# Autodesk Inventor assembly: Pogo_Set2
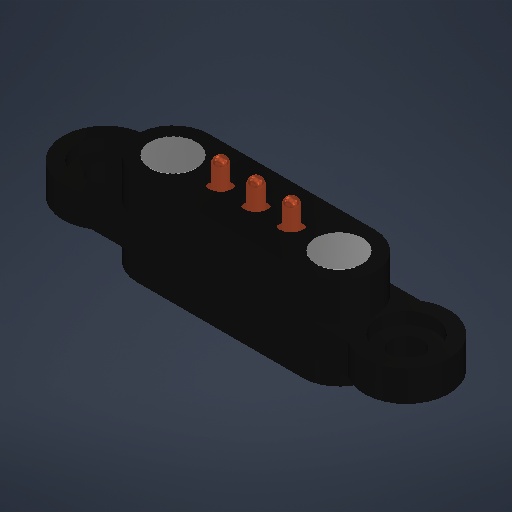
[picture p0: Inventor's stored thumbnail of the model, 512x512]
Saved by Autodesk Inventor 2026 (Build 300175000, 175)
## iProperties
Created: 2025-04-18
Part Number: Pogo_Set2
Document SubType Name: Assembly
Designer: ct_vi
Author: ct_vi
## Documents named in this file (5)
- C:\Users\ct_vi\Documents\Capstone_Research_3D_Files\Pogo_Set2.iam
- C:\Users\ct_vi\Documents\Capstone_Research_3D_Files\Pogo2.ipt
- C:\Users\ct_vi\Documents\Capstone_Research_3D_Files\Pogo_Pin2.ipt
- Pogo_Pin2.ipt
- C:\Users\ct_vi\Documents\Capstone_Research_3D_Files\Magnet_Pogo2.ipt
## Components (4 placed, 3 different names)
1. Pogo_Pin2:1 — Mate:1, Mate:2, Mate:3
2. Pogo2:2 — Mate:1, Mate:2, Mate:3, Mate:4, Mate:5, Flush:1, Flush:2
3. Magnet_Pogo2:1 — Mate:5, Flush:1
4. Magnet_Pogo2:2 — Mate:4, Flush:2
## Relationships (7: Mate 5, Flush 2)
- Mate:1: Pogo_Pin2:1 ↔ Pogo2:2
- Mate:2: Pogo_Pin2:1 ↔ Pogo2:2
- Mate:3: Pogo_Pin2:1 ↔ Pogo2:2
- Mate:4: Pogo2:2 ↔ Magnet_Pogo2:2
- Mate:5: Pogo2:2 ↔ Magnet_Pogo2:1
- Flush:1: Pogo2:2 ↔ Magnet_Pogo2:1
- Flush:2: Pogo2:2 ↔ Magnet_Pogo2:2
